# Autodesk Inventor assembly: Throttle
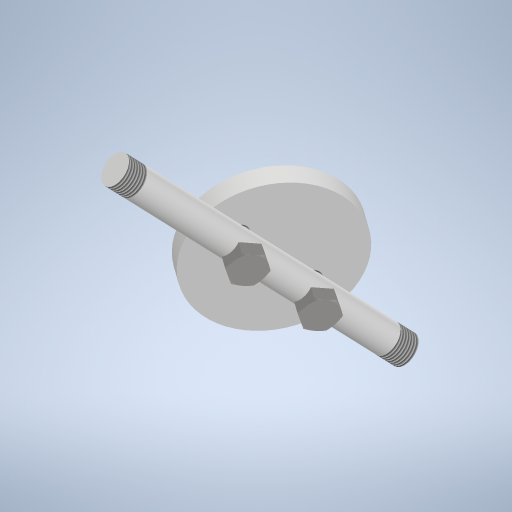
[picture p0: Inventor's stored thumbnail of the model, 512x512]
Saved by Autodesk Inventor 2023 (Build 270158000, 158)
## iProperties
Created: 2023-07-26
Part Number: Throttle
Document SubType Name: Assembly
Designer: User
Author: User
## Documents named in this file (5)
- C:\Users\User\Desktop\BIANCA\SCHOOL WORK\INVENTOR 2023\CRUISE CONTROL\Throttle.iam
- C:\Users\User\Documents\Inventor\Content Center Files\R2023\en-US\ANSI B18.2.3.5M\ANSI B18.2.3.5M - M10 x 1.5 x 35.ipt
- C:\Users\User\Desktop\BIANCA\SCHOOL WORK\INVENTOR 2023\CRUISE CONTROL\shaft2.ipt
- C:\Users\User\Desktop\BIANCA\SCHOOL WORK\INVENTOR 2023\CRUISE CONTROL\Throttle.ipt
- C:\Users\User\Documents\Inventor\Content Center Files\R2023\en-US\ANSI B 18.2.4.1 M(1)\ANSI B 18.2.4.1 M - M10 x 1.5Style 1.ipt
## Components (6 placed, 4 different names)
1. Hex Bolt - Metric M10 x 1.5 x 35:1 — Rigid:1, Insert:1
2. shaft2:1 — Rigid:1, Rigid:2
3. Throttle:1 — Insert:1, Rigid:3, Rigid:4
4. Hex Bolt - Metric M10 x 1.5 x 35:2 — Rigid:2
5. Hex Nut Metric M10 x 1.5:1 — Rigid:4
6. Hex Nut Metric M10 x 1.5:2 — Rigid:3
## Relationships (5: WeldJoint 4, Insert 1)
- Rigid:1 [WeldJoint]: Hex Bolt - Metric M10 x 1.5 x 35:1 ↔ shaft2:1
- Rigid:2 [WeldJoint]: shaft2:1 ↔ Hex Bolt - Metric M10 x 1.5 x 35:2
- Insert:1 (-20 mm): Hex Bolt - Metric M10 x 1.5 x 35:1 ↔ Throttle:1
- Rigid:3 [WeldJoint]: Throttle:1 ↔ Hex Nut Metric M10 x 1.5:2
- Rigid:4 [WeldJoint]: Throttle:1 ↔ Hex Nut Metric M10 x 1.5:1
